# Autodesk Inventor assembly: 組合彈珠檯
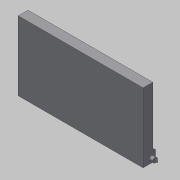
[picture p0: Inventor's stored thumbnail of the model, 180x180]
Saved by Autodesk Inventor 2018 (Build 220112000, 112)
## iProperties
Created: 2020-12-16
Part Number: 組合彈珠檯
Material: 一般
Document SubType Name: Assembly
Designer: 王鼎鈞
Author: 王鼎鈞
## Documents named in this file (4)
- C:\Users\王鼎鈞\Desktop\組合彈珠檯.iam
- C:\Users\王鼎鈞\Desktop\彈珠檯完成品.ipt
- C:\Users\王鼎鈞\Desktop\彈珠檯啟動桿.ipt
- C:\Users\王鼎鈞\Desktop\彈珠檯球.ipt
## Components (3 placed, 3 different names)
1. 彈珠檯完成品:1 — 貼合:1, 相切:1, 貼合:2
2. 彈珠檯啟動桿:1 — 貼合:1, 貼合:2
3. 彈珠檯球:1 — 相切:1
## Relationships (3: Mate 2, Tangent 1)
- 貼合:1 [Mate]: 彈珠檯完成品:1 ↔ 彈珠檯啟動桿:1
- 相切:1 [Tangent]: 彈珠檯完成品:1 ↔ 彈珠檯球:1
- 貼合:2 [Mate]: 彈珠檯完成品:1 ↔ 彈珠檯啟動桿:1
